# Autodesk Inventor assembly: Sled
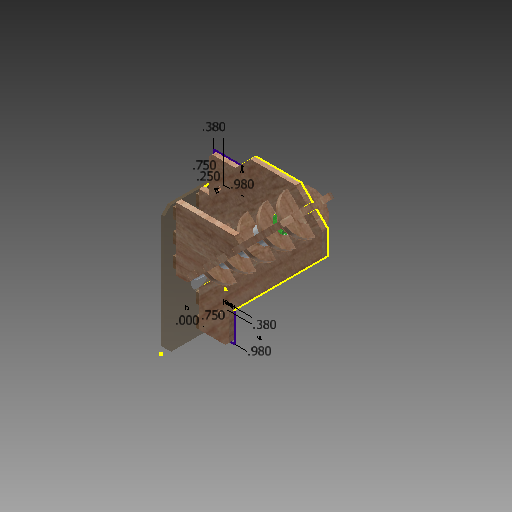
[picture p0: Inventor's stored thumbnail of the model, 512x512]
Saved by Autodesk Inventor 2019 (Build 230136000, 136)
## iProperties
Created: 2019-01-14
Part Number: Sled
Document SubType Name: Assembly
Designer: nxgam
Author: nxgam
## Documents named in this file (5)
- C:\Users\nxgam\Documents\CAD\Inventor\DiscoDraw\Sled.iam
- C:\Users\nxgam\Documents\CAD\Inventor\DiscoDraw\Sleigh.ipt
- C:\Users\nxgam\Documents\CAD\Inventor\DiscoDraw\MarkerHolder.iam
- C:\Users\nxgam\Documents\CAD\Inventor\DiscoDraw\SledSideSupport.ipt
- C:\Users\nxgam\Documents\CAD\Inventor\DiscoDraw\BeltMount.ipt
## Components (6 placed, 4 different names)
1. Sleigh:1 — Mate:1, Mate:2, Mate:3, Mate:4, Mate:5, Mate:6, Mate:7, Angle:1
2. MarkerHolder:1 [sub-assembly] — Mate:1, Mate:2, Mate:3, Mate:8, Mate:9, Mate:10, Mate:11
3. SledSideSupport:1 — Flush:1, Flush:2, Mate:5, Flush:3
4. SledSideSupport:2 — Flush:1, Flush:2, Mate:4, Mate:6, Flush:3, Mate:7
5. BeltMount:1 — Flush:4, Flush:5, Mate:10, Mate:11
6. BeltMount:2 — Mate:8, Angle:1, Flush:4, Flush:5, Mate:9
## Relationships (17: Mate 11, Flush 5, Angle 1)
- Mate:1: Sleigh:1 ↔ MarkerHolder:1
- Mate:2: Sleigh:1 ↔ MarkerHolder:1
- Mate:3: Sleigh:1 ↔ MarkerHolder:1
- Flush:1: SledSideSupport:1 ↔ SledSideSupport:2
- Flush:2: SledSideSupport:1 ↔ SledSideSupport:2
- Mate:4: Sleigh:1 ↔ SledSideSupport:2
- Mate:5: Sleigh:1 ↔ SledSideSupport:1
- Mate:6: Sleigh:1 ↔ SledSideSupport:2
- Flush:3: SledSideSupport:1 ↔ SledSideSupport:2
- Mate:7: Sleigh:1 ↔ SledSideSupport:2
- Mate:8: MarkerHolder:1 ↔ BeltMount:2
- Angle:1 (90 deg): Sleigh:1 ↔ BeltMount:2
- Flush:4: BeltMount:1 ↔ BeltMount:2
- Flush:5: BeltMount:1 ↔ BeltMount:2
- Mate:9: MarkerHolder:1 ↔ BeltMount:2
- Mate:10: MarkerHolder:1 ↔ BeltMount:1
- Mate:11: MarkerHolder:1 ↔ BeltMount:1
